# Autodesk Inventor assembly: 2f2
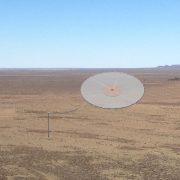
[picture p0: Inventor's stored thumbnail of the model, 180x180]
Saved by Autodesk Inventor 2014 SP1 (Build 180222100, 222)
## iProperties
Company: HERA Project
Created: 2013-06-27
Part Number: 2f2
Document SubType Name: Assembly
Designer: David DeBoer
Description: Feed backplane support assembly
Author: David DeBoer
Title: Feed backplane support
## Documents named in this file (9)
- C:\Users\Dave\Desktop\hera-cad\feed\bpScreenAssembly.iam
- C:\Users\Dave\Desktop\hera-cad\feed\bpSupArm.ipt
- C:\Users\Dave\Desktop\hera-cad\smallParts\pvc_T_0.75in.ipt
- C:\Users\Dave\Desktop\hera-cad\feed\bpSupArc.ipt
- C:\Users\Dave\Desktop\hera-cad\feed\bpScreen.ipt
- C:\Users\Dave\Desktop\hera-cad\feed\bpCylinder.ipt
- C:\Users\Dave\Desktop\hera-cad\jigs\bpSparJig.ipt
- C:\Users\Dave\Desktop\hera-cad\feed\bpSupVertArm.ipt
- C:\Users\Dave\Desktop\hera-cad\smallParts\angleBracketB.ipt
## Components (25 placed, 8 different names)
1. bpSparJig:1 — Insert:6, Insert:7, Insert:8
2. bpScreen:1 — Insert:8, Angle:3, Insert:13
3. bpSupVertArm:1 — Insert:11, Angle:7, Insert:14, Angle:8
4. pvc_T_0.75in:7 — Insert:11, Angle:6, Insert:12, Angle:0
5. bpSupArc:7 — Insert:12, Angle:7
6. bpCylinder:1 — Insert:13
7. angleBracketB:1 — Insert:14, Angle:8, Angle:0
8. bpSupArm:1 — Insert:4, Angle:1, Angle:2, Insert:6, Insert:7
9. pvc_T_0.75in:1 — Insert:4, Insert:5, Angle:2
10. bpSupArc:1 — Insert:5, Angle:1
11. bpSupArm:2
12. pvc_T_0.75in:2 — Angle:6
13. bpSupArc:2
14. bpSupArm:3
15. pvc_T_0.75in:3 — Angle:3
16. bpSupArc:3
17. bpSupArm:4
18. pvc_T_0.75in:4
19. bpSupArc:4
20. bpSupArm:5
21. pvc_T_0.75in:5
22. bpSupArc:5
23. bpSupArm:6
24. pvc_T_0.75in:6
25. bpSupArc:6
## Component patterns: (6 elements, first: bpSupArm:1 + pvc_T_0.75in:1 + bpSupArc:1)
## Relationships (16: Insert 9, Angle 7)
- Insert:4 (-12.7 mm): bpSupArm:1 ↔ pvc_T_0.75in:1
- Insert:5: pvc_T_0.75in:1 ↔ bpSupArc:1
- Angle:1 (30 deg): bpSupArm:1 ↔ bpSupArc:1
- Angle:2 (90 deg): bpSupArm:1 ↔ pvc_T_0.75in:1
- Insert:6: bpSparJig:1 ↔ bpSupArm:1
- Insert:7: bpSparJig:1 ↔ bpSupArm:1
- Insert:8 (25.4 mm): bpSparJig:1 ↔ bpScreen:1
- Angle:3 (180 deg): bpScreen:1 ↔ pvc_T_0.75in:3
- Insert:11 (-12.7 mm): bpSupVertArm:1 ↔ pvc_T_0.75in:7
- Angle:6 (0 deg): pvc_T_0.75in:7 ↔ pvc_T_0.75in:2
- Insert:12 (-12.7 mm): pvc_T_0.75in:7 ↔ bpSupArc:7
- Angle:7 (180 deg): bpSupVertArm:1 ↔ bpSupArc:7
- Insert:13: bpScreen:1 ↔ bpCylinder:1
- Insert:14: bpSupVertArm:1 ↔ angleBracketB:1
- Angle:8 (180 deg): bpSupVertArm:1 ↔ angleBracketB:1
- Angle:0 (0 deg): pvc_T_0.75in:7 ↔ angleBracketB:1
